# Autodesk Inventor assembly: Фильтр D1000
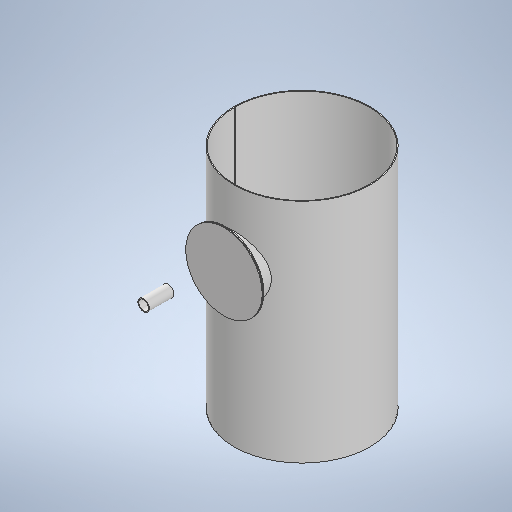
[picture p0: Inventor's stored thumbnail of the model, 512x512]
Saved by Autodesk Inventor 2025 (Build 290162010, 162A)
## iProperties
Created: 2025-02-12
Part Number: Фильтр D1000
Document SubType Name: Assembly
Designer: pokla
Author: pokla
## Documents named in this file (7)
- C:\Users\pokla\Desktop\Работа Акватроник\Фильтры напорные\Фильтр D1000.iam
- C:\Users\pokla\Desktop\Работа Акватроник\Фильтры напорные\Стенка фильтра D1000.ipt
- C:\Users\pokla\Desktop\Работа Акватроник\Фильтры напорные\Размеры D1000.ipt
- C:\Users\pokla\Desktop\Работа Акватроник\Фильтры напорные\Ревиз. окно фильтра D1000.ipt
- C:\Users\pokla\Desktop\Работа Акватроник\Фильтры напорные\Кольцо заглушки ревиз. окна фильтра D1000.ipt
- C:\Users\pokla\Desktop\Работа Акватроник\Фильтры напорные\Заглушка ревиз. окна фильтра D1000.ipt
- C:\Users\pokla\Desktop\Работа Акватроник\Фильтры напорные\Труба подключения фильтра D1000.ipt
## Components (7 placed, 6 different names)
1. Размеры D1000:1
2. Стенка фильтра D1000:1 — Mate:1, Flush:1
3. Ревиз. окно фильтра D1000:1 — Mate:1, Flush:1, Flush:2, Rigid:2
4. Кольцо заглушки ревиз. окна фильтра D1000:1 — Rigid:1, Rigid:2, Rigid:3
5. Кольцо заглушки ревиз. окна фильтра D1000:2 — Rigid:1
6. Заглушка ревиз. окна фильтра D1000:1 — Rigid:3
7. Труба подключения фильтра D1000:1
## Relationships (6: WeldJoint 3, Flush 2, Mate 1)
- Mate:1: Стенка фильтра D1000:1 ↔ Ревиз. окно фильтра D1000:1
- Flush:1 (495 mm): Стенка фильтра D1000:1 ↔ Ревиз. окно фильтра D1000:1
- Flush:2: Ревиз. окно фильтра D1000:1
- Rigid:1 [WeldJoint]: Кольцо заглушки ревиз. окна фильтра D1000:1 ↔ Кольцо заглушки ревиз. окна фильтра D1000:2
- Rigid:2 [WeldJoint]: Ревиз. окно фильтра D1000:1 ↔ Кольцо заглушки ревиз. окна фильтра D1000:1
- Rigid:3 [WeldJoint]: Кольцо заглушки ревиз. окна фильтра D1000:1 ↔ Заглушка ревиз. окна фильтра D1000:1
